# Autodesk Inventor assembly: 組合
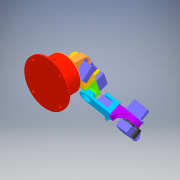
[picture p0: Inventor's stored thumbnail of the model, 180x180]
Saved by Autodesk Inventor 2017 (Build 210142000, 142)
## iProperties
Part Number: 組合
Material: 一般
Document SubType Name: Assembly
Designer: Brian
Mass: 1020.2 g
Surface Area: 2193.1 cm^2
Volume: 598.179 cm^3
Density: 1.70551 g/cm^3
Author: Brian
## Documents named in this file (7)
- E:\Brian\檔案\機械手臂\組合.iam
- E:\Brian\檔案\機械手臂\底座.ipt
- E:\Brian\檔案\機械手臂\MG996 伺服馬達.ipt
- E:\Brian\檔案\機械手臂\第一關節.ipt
- E:\Brian\檔案\機械手臂\第一臂-1.ipt
- E:\Brian\檔案\機械手臂\第一臂-2.ipt
- E:\Brian\檔案\機械手臂\腕-2.ipt
## Components (14 placed, 12 different names)
1. 底座:1 — 貼合:3, 貼合:4, 貼合:5, 貼合:8
2. bottonSpin — 貼合:3, 貼合:4, 貼合:5, 貼合:9
3. 第一關節:1 — 貼合:6, 齊平:1, 貼合:8, 貼合:9, 貼合:10, 貼合:32
4. bottonRotate — 貼合:6, 齊平:1, 貼合:13, 貼合:32
5. 第一臂-1:1 — 貼合:10, 貼合:12, 齊平:2, 貼合:13, 角度:1
6. secSpin — 貼合:12, 齊平:2, 角度:1, 貼合:14, 貼合:15
7. 第一臂-2:1 — 貼合:14, 貼合:15, 齊平:3, 貼合:16, 貼合:17
8. secRotate — 齊平:3, 貼合:16, 貼合:17, 貼合:23, 貼合:24
9. 第一臂-1:2 — 貼合:23, 貼合:24
10. armSpin
11. 第一臂-2:2 — 貼合:25, 貼合:26, 貼合:28
12. armRotate — 貼合:25, 貼合:26, 貼合:27
13. 腕-2:1 — 貼合:27, 貼合:28, 貼合:29, 貼合:30, 貼合:31
14. MG996 伺服馬達:7 — 貼合:29, 貼合:30, 貼合:31
## Relationships (33: Mate 26, Flush 5, Angle 2)
- 貼合:3 [Mate]: 底座:1 ↔ bottonSpin
- 貼合:4 [Mate]: 底座:1 ↔ bottonSpin
- 貼合:5 [Mate]: 底座:1 ↔ bottonSpin
- 貼合:6 [Mate]: 第一關節:1 ↔ bottonRotate
- 齊平:1 [Flush]: 第一關節:1 ↔ bottonRotate
- 貼合:8 [Mate]: 底座:1 ↔ 第一關節:1
- 貼合:9 [Mate]: bottonSpin ↔ 第一關節:1
- 貼合:10 [Mate]: 第一關節:1 ↔ 第一臂-1:1
- 貼合:12 [Mate]: 第一臂-1:1 ↔ secSpin
- 齊平:2 [Flush]: 第一臂-1:1 ↔ secSpin
- 貼合:13 [Mate]: bottonRotate ↔ 第一臂-1:1
- 角度:1 [Angle] (180 deg): 第一臂-1:1 ↔ secSpin
- 貼合:14 [Mate]: secSpin ↔ 第一臂-2:1
- 貼合:15 [Mate]: secSpin ↔ 第一臂-2:1
- 齊平:3 [Flush]: 第一臂-2:1 ↔ secRotate
- 貼合:16 [Mate]: 第一臂-2:1 ↔ secRotate
- 貼合:17 [Mate]: 第一臂-2:1 ↔ secRotate
- [Mate]: 第一臂-1:2 ↔ armSpin
- [Flush]: 第一臂-1:2 ↔ armSpin
- [Angle] (180 deg): 第一臂-1:2 ↔ armSpin
- [Mate]: armSpin ↔ 第一臂-2:2
- [Mate]: armSpin ↔ 第一臂-2:2
- [Flush]: 第一臂-2:2 ↔ armRotate
- 貼合:23 [Mate]: secRotate ↔ 第一臂-1:2
- 貼合:24 [Mate]: secRotate ↔ 第一臂-1:2
- 貼合:25 [Mate]: 第一臂-2:2 ↔ armRotate
- 貼合:26 [Mate]: 第一臂-2:2 ↔ armRotate
- 貼合:27 [Mate]: armRotate ↔ 腕-2:1
- 貼合:28 [Mate]: 第一臂-2:2 ↔ 腕-2:1
- 貼合:29 [Mate]: 腕-2:1 ↔ MG996 伺服馬達:7
- 貼合:30 [Mate]: 腕-2:1 ↔ MG996 伺服馬達:7
- 貼合:31 [Mate]: 腕-2:1 ↔ MG996 伺服馬達:7
- 貼合:32 [Mate]: 第一關節:1 ↔ bottonRotate
## Named parameters: d32_d16 = 0 mm, d33_d17 = 0 mm, d34_d21 = 180 deg, d35_d22 = 0 mm, d36_d23 = 0 mm, d37_d25 = 0 mm
